# Autodesk Inventor assembly: 3614-0014-0096 assembly
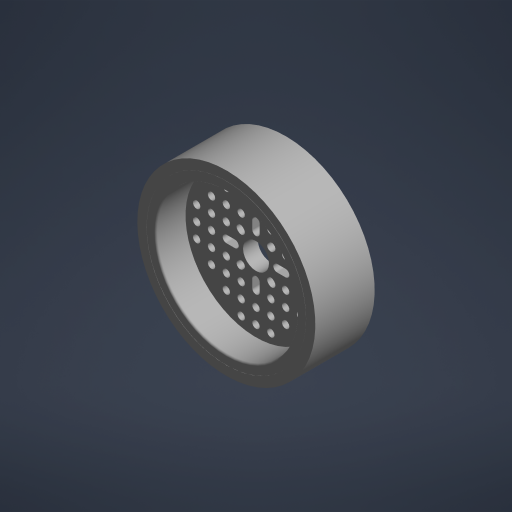
[picture p0: Inventor's stored thumbnail of the model, 512x512]
Saved by Autodesk Inventor 2023 (Build 270158000, 158)
## iProperties
Created: 2020-12-15
Part Number: 3614-0014-0096 assembly
Description: STEP AP203
Document SubType Name: Assembly
Designer: izack
Sending System: SolidWorks 2016
Preprocessor: SwSTEP 2.0
Title: 3614-0014-0096 assembly.STEP
Revision Number: ANY
## Documents named in this file (3)
- G:\CAD Modeling\Private Robotics\Custom Tryhard Robot\Drivetrain\Swerve Module Parts\96mm GoBilda Traction Wheel.iam
- G:\CAD Modeling\Private Robotics\Custom Tryhard Robot\Drivetrain\Swerve Module Parts\96mm Gobilda Traction Wheel Parts\3614-0014-0096 wheel.ipt
- G:\CAD Modeling\Private Robotics\Custom Tryhard Robot\Drivetrain\Swerve Module Parts\96mm Gobilda Traction Wheel Parts\3614-0014-0096 wheel ring.ipt
## Components (2 placed, 2 different names)
1. 3614-0014-0096 wheel_1 — Rigid:1
2. 3614-0014-0096 wheel ring_2 — Rigid:1
## Relationships (1: WeldJoint 1)
- Rigid:1 [WeldJoint]: 3614-0014-0096 wheel_1 ↔ 3614-0014-0096 wheel ring_2
